# Autodesk Inventor assembly: Microdrive_Compact_Body
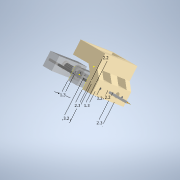
[picture p0: Inventor's stored thumbnail of the model, 180x180]
Saved by Autodesk Inventor 2020 (Build 240168000, 168)
## iProperties
Created: 2019-11-04
Part Number: Microdrive_Compact_Body
Document SubType Name: Assembly
Designer: Knowblesse
Author: Knowblesse
## Documents named in this file (10)
- C:\VCF\Microdrive\Compact\Microdrive_Compact_Body.iam
- C:\VCF\Microdrive\Compact\Bot.ipt
- C:\VCF\Microdrive\Compact\Top.ipt
- C:\VCF\Microdrive\Nut.ipt
- C:\VCF\Microdrive\Compact\23G_Pillar.ipt
- C:\VCF\Microdrive\Compact\Screw.ipt
- C:\VCF\Microdrive\Compact\23G_Holder.ipt
- C:\VCF\Microdrive\Compact\Polyimide.ipt
- C:\VCF\Microdrive\Compact\Tetrode.ipt
- C:\VCF\Microdrive\Compact\Body.ipt
## Components (10 placed, 9 different names)
1. Bot:1 — 메이트:7, 메이트:8, 강체:1
2. Top:1 — 회전:2, 메이트:2, 회전:4, 메이트:4, 회전:5, 회전:7
3. Nut:1 — 회전:2
4. 23G_Pillar:1 — 메이트:2, 회전:4, 메이트:8
5. 23G_Pillar:2 — 메이트:4, 회전:5, 메이트:7, 강체:4
6. Screw:1 — 회전:7, 메이트:9
7. 23G_Holder:1 — 강체:1, 강체:2
8. Polyimide:1 — 강체:2, 강체:3
9. Tetrode:1 — 강체:3
10. Body:1 — 메이트:9, 강체:4
## Relationships (13: Mate 5, RevoluteJoint 4, WeldJoint 4)
- 회전:2 [RevoluteJoint]: Top:1 ↔ Nut:1
- 메이트:2 [Mate]: Top:1 ↔ 23G_Pillar:1
- 회전:4 [RevoluteJoint]: Top:1 ↔ 23G_Pillar:1
- 메이트:4 [Mate]: Top:1 ↔ 23G_Pillar:2
- 회전:5 [RevoluteJoint]: Top:1 ↔ 23G_Pillar:2
- 회전:7 [RevoluteJoint]: Top:1 ↔ Screw:1
- 메이트:7 [Mate]: Bot:1 ↔ 23G_Pillar:2
- 메이트:8 [Mate]: Bot:1 ↔ 23G_Pillar:1
- 강체:1 [WeldJoint] (-0.5 mm): Bot:1 ↔ 23G_Holder:1
- 강체:2 [WeldJoint] (0.5 mm): 23G_Holder:1 ↔ Polyimide:1
- 강체:3 [WeldJoint] (0.5 mm): Polyimide:1 ↔ Tetrode:1
- 메이트:9 [Mate]: Screw:1 ↔ Body:1
- 강체:4 [WeldJoint]: 23G_Pillar:2 ↔ Body:1
